# Autodesk Inventor assembly: 42146-36
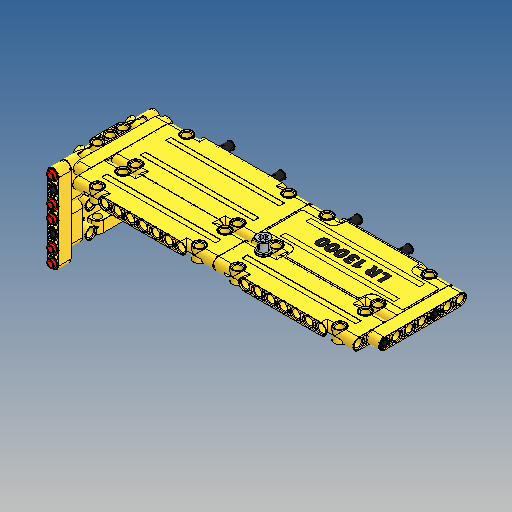
[picture p0: Inventor's stored thumbnail of the model, 512x512]
Saved by Autodesk Inventor 2025 (Build 290162010, 162A)
## iProperties
Created: 2024-12-07
Part Number: 42146-36
Material: Generisch
Document SubType Name: Assembly
Designer: hp.muther
Author: hp.muther
## Documents named in this file (11)
- D:\Inventor\Projekte\Muther\LEGO Technic\LEGO Technik - Raupenkran LR 13000 (42146)\42146-36.iam
- D:\Inventor\Projekte\Muther\LEGO Technic\LEGO Pieces\Paneelen\64782-Yellow.ipt
- D:\Inventor\Projekte\Muther\LEGO Technic\LEGO Pieces\Paneelen\15458-Yellow.ipt
- D:\Inventor\Projekte\Muther\LEGO Technic\LEGO Pieces\Lochbalken\32524-Yellow.ipt
- D:\Inventor\Projekte\Muther\LEGO Technic\LEGO Pieces\Pin's\2780-Black.ipt
- D:\Inventor\Projekte\Muther\LEGO Technic\LEGO Pieces\Pin's\6558-Blue.ipt
- D:\Inventor\Projekte\Muther\LEGO Technic\LEGO Pieces\Pin's\4274-Red.ipt
- D:\Inventor\Projekte\Muther\LEGO Technic\LEGO Pieces\Paneelen\71709-Yellow.ipt
- D:\Inventor\Projekte\Muther\LEGO Technic\LEGO Pieces\Winkel\32526-Yellow.ipt
- D:\Inventor\Projekte\Muther\LEGO Technic\LEGO Pieces\Pin's\32054-LtBluishGray.ipt
- D:\Inventor\Projekte\Muther\LEGO Technic\LEGO Technik - Raupenkran LR 13000 (42146)\42146_64782_1.ipt
## Components (38 placed, 10 different names)
1. 15458-Yellow:2 — Einfügen:12, Passend:3, Einfügen:13, Passend:5
2. 42146_64782_1:2 — Einfügen:1, Einfügen:2, Einfügen:5, Einfügen:8, Einfügen:10, Einfügen:11, Einfügen:36, Einfügen:37
3. 15458-Yellow:1 — Einfügen:5, Passend:1, Passend:2, Einfügen:9, Einfügen:13, Einfügen:33
4. 32524-Yellow:1 — Einfügen:6, Einfügen:7, Einfügen:8
5. 2780-Black:1 — Einfügen:1
6. 2780-Black:2 — Einfügen:2, Passend:1
7. 6558-Blue:1 — Einfügen:14, Passend:8
8. 6558-Blue:2 — Einfügen:15, Passend:5
9. 2780-Black:3 — Einfügen:6
10. 2780-Black:4 — Einfügen:7, Passend:2
11. 2780-Black:5 — Einfügen:9
12. 64782-Yellow:1 — Einfügen:12, Passend:4, Einfügen:16, Einfügen:34, Einfügen:35
13. 2780-Black:6 — Passend:3
14. 2780-Black:7
15. 2780-Black:8 — Einfügen:11, Passend:4
16. 2780-Black:9 — Einfügen:10
17. 32524-Yellow:2 — Einfügen:14, Einfügen:15, Einfügen:16, Einfügen:32
18. 4274-Red:1 — Einfügen:21
19. 4274-Red:2 — Einfügen:19
20. 4274-Red:3 — Einfügen:20
21. 4274-Red:4 — Einfügen:18
22. 4274-Red:5 — Einfügen:17
23. 2780-Black:10 — Einfügen:22, Passend:6
24. 2780-Black:11 — Einfügen:23
25. 2780-Black:12 — Einfügen:25
26. 2780-Black:13 — Einfügen:24
27. 32524-Yellow:3 — Einfügen:17, Einfügen:18, Einfügen:19, Einfügen:20, Einfügen:21, Einfügen:22, Einfügen:23, Einfügen:27
28. 71709-Yellow:1 — Einfügen:24, Einfügen:25, Einfügen:26, Passend:6, Einfügen:29, Einfügen:30
29. 71709-Yellow:2 — Einfügen:26, Einfügen:27, Einfügen:28, Einfügen:32, Passend:8
30. 32526-Yellow:1 — Einfügen:30, Passend:7, Einfügen:31
31. 2780-Black:14 — Einfügen:28, Passend:7
32. 2780-Black:15 — Einfügen:29
33. 32054-LtBluishGray:1 — Einfügen:31
34. 32054-LtBluishGray:2 — Einfügen:33
35. 2780-Black:16 — Einfügen:34
36. 2780-Black:17 — Einfügen:35
37. 2780-Black:18 — Einfügen:36
38. 2780-Black:19 — Einfügen:37
## Relationships (45: Insert 37, Mate 8)
- Einfügen:1 [Insert]: 42146_64782_1:2 ↔ 2780-Black:1
- Einfügen:2 [Insert]: 42146_64782_1:2 ↔ 2780-Black:2
- [Insert]: 64782-Yellow:1 ↔ 2780-Black:6
- [Insert]: 64782-Yellow:1 ↔ 2780-Black:7
- Einfügen:5 [Insert]: 42146_64782_1:2 ↔ 15458-Yellow:1
- Passend:1 [Mate]: 15458-Yellow:1 ↔ 2780-Black:2
- Einfügen:6 [Insert]: 32524-Yellow:1 ↔ 2780-Black:3
- Einfügen:7 [Insert]: 32524-Yellow:1 ↔ 2780-Black:4
- Einfügen:8 [Insert]: 42146_64782_1:2 ↔ 32524-Yellow:1
- Passend:2 [Mate]: 15458-Yellow:1 ↔ 2780-Black:4
- Einfügen:9 [Insert]: 15458-Yellow:1 ↔ 2780-Black:5
- Einfügen:10 [Insert]: 42146_64782_1:2 ↔ 2780-Black:9
- Einfügen:11 [Insert]: 42146_64782_1:2 ↔ 2780-Black:8
- Einfügen:12 [Insert]: 15458-Yellow:2 ↔ 64782-Yellow:1
- Passend:3 [Mate]: 15458-Yellow:2 ↔ 2780-Black:6
- Einfügen:13 [Insert]: 15458-Yellow:2 ↔ 15458-Yellow:1
- Passend:4 [Mate]: 64782-Yellow:1 ↔ 2780-Black:8
- Einfügen:14 [Insert]: 6558-Blue:1 ↔ 32524-Yellow:2
- Einfügen:15 [Insert]: 6558-Blue:2 ↔ 32524-Yellow:2
- Einfügen:16 [Insert]: 64782-Yellow:1 ↔ 32524-Yellow:2
- Passend:5 [Mate]: 15458-Yellow:2 ↔ 6558-Blue:2
- Einfügen:17 [Insert]: 4274-Red:5 ↔ 32524-Yellow:3
- Einfügen:18 [Insert]: 4274-Red:4 ↔ 32524-Yellow:3
- Einfügen:19 [Insert]: 4274-Red:2 ↔ 32524-Yellow:3
- Einfügen:20 [Insert]: 4274-Red:3 ↔ 32524-Yellow:3
- Einfügen:21 [Insert]: 4274-Red:1 ↔ 32524-Yellow:3
- Einfügen:22 [Insert]: 2780-Black:10 ↔ 32524-Yellow:3
- Einfügen:23 [Insert]: 2780-Black:11 ↔ 32524-Yellow:3
- Einfügen:24 [Insert]: 2780-Black:13 ↔ 71709-Yellow:1
- Einfügen:25 [Insert]: 2780-Black:12 ↔ 71709-Yellow:1
- Einfügen:26 [Insert]: 71709-Yellow:1 ↔ 71709-Yellow:2
- Einfügen:27 [Insert]: 32524-Yellow:3 ↔ 71709-Yellow:2
- Passend:6 [Mate]: 2780-Black:10 ↔ 71709-Yellow:1
- Einfügen:28 [Insert]: 71709-Yellow:2 ↔ 2780-Black:14
- Einfügen:29 [Insert]: 71709-Yellow:1 ↔ 2780-Black:15
- Einfügen:30 [Insert]: 71709-Yellow:1 ↔ 32526-Yellow:1
- Passend:7 [Mate]: 32526-Yellow:1 ↔ 2780-Black:14
- Einfügen:31 [Insert]: 32526-Yellow:1 ↔ 32054-LtBluishGray:1
- Einfügen:32 [Insert]: 32524-Yellow:2 ↔ 71709-Yellow:2
- Passend:8 [Mate]: 6558-Blue:1 ↔ 71709-Yellow:2
- Einfügen:33 [Insert]: 15458-Yellow:1 ↔ 32054-LtBluishGray:2
- Einfügen:34 [Insert]: 64782-Yellow:1 ↔ 2780-Black:16
- Einfügen:35 [Insert]: 64782-Yellow:1 ↔ 2780-Black:17
- Einfügen:36 [Insert]: 42146_64782_1:2 ↔ 2780-Black:18
- Einfügen:37 [Insert]: 42146_64782_1:2 ↔ 2780-Black:19
## Named parameters: d2_d0 = 0 mm, d3_d1 = 0 mm
